# Autodesk Inventor assembly: Drive2
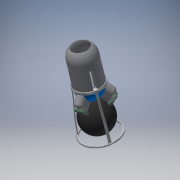
[picture p0: Inventor's stored thumbnail of the model, 180x180]
Saved by Autodesk Inventor 2019.1 (Build 231200000, 200)
## iProperties
Created: 2018-06-30
Part Number: Drive2
Material: Generisch
Document SubType Name: Assembly
Designer: JochenAlt
Author: JochenAlt
## Documents named in this file (10)
- D:\Projects\Ondine\CAD\Drive.iam
- D:\Projects\Ondine\CAD\Sphere.ipt
- D:\Projects\Ondine\CAD\DriveChain.iam
- D:\Projects\Ondine\CAD\Spindle\SpindleWithGear.ipt
- D:\Projects\Ondine\CAD\Spindle\Spindle.ipt
- D:\Projects\Ondine\CAD\Bearings\W 61700 X-2RS1.iam
- D:\Projects\Ondine\CAD\SpindleMotor.iam
- D:\Projects\Ondine\CAD\PCB\ControllerPCBHolder.ipt
- D:\Projects\Ondine\CAD\PCB\MotorController.ipt
- D:\Projects\Ondine\CAD\Form.iam
## Components (18 placed, 8 different names)
1. Sphere:1 — Passend:38, Passend:61, Passend:121, Passend:122
2. DriveChain:1 [sub-assembly] — Passend:61, Passend:95, Passend:103, Passend:104, Passend:105, Passend:110, Passend:115, Passend:121, Passend:122, Passend:127, Passend:130
3. DriveChain:2 [sub-assembly] — Passend:84, Passend:87, Passend:95, Passend:99, Passend:109, Passend:110, Passend:111, Passend:112, Passend:116
4. DriveChain:3 [sub-assembly] — Passend:89, Passend:93, Passend:103, Passend:104, Passend:111, Passend:113, Passend:128
5. Spindle:1 — Passend:66, Passend:72, Passend:77, Fluchtend:1
6. Spindle:2 — Passend:67, Passend:75, Passend:76, Passend:93
7. Spindle:3 — Passend:73, Passend:114, Passend:117, Passend:129
8. W 61700 X-2RS1:1 [sub-assembly] — Passend:66, Passend:112
9. W 61700 X-2RS1:2 [sub-assembly]
10. W 61700 X-2RS1:3 [sub-assembly] — Passend:67, Passend:113
11. W 61700 X-2RS1:4 [sub-assembly] — Passend:72, Passend:77, Passend:87, Passend:109
12. W 61700 X-2RS1:5 [sub-assembly] — Passend:75, Passend:76, Passend:89
13. W 61700 X-2RS1:6 [sub-assembly] — Passend:73, Passend:116, Passend:117
14. SpindleMotor:1 [sub-assembly] — Passend:84, Fluchtend:1
15. PCBHolder:1 — Passend:99, Passend:105, Passend:125, Passend:126, Passend:127, Passend:128
16. MotorController:1 — Passend:125, Passend:126
17. W 61700 X-2RS1:7 [sub-assembly] — Passend:114, Passend:115
18. Form:1 [sub-assembly] — Passend:129, Passend:130
## Relationships (36: Mate 35, Flush 1)
- Passend:38 [Mate]: Sphere:1
- Passend:61 [Mate] (89 mm): Sphere:1 ↔ DriveChain:1
- Passend:66 [Mate]: Spindle:1 ↔ W 61700 X-2RS1:1
- Passend:67 [Mate]: Spindle:2 ↔ W 61700 X-2RS1:3
- Passend:72 [Mate]: Spindle:1 ↔ W 61700 X-2RS1:4
- Passend:73 [Mate]: Spindle:3 ↔ W 61700 X-2RS1:6
- Passend:75 [Mate]: Spindle:2 ↔ W 61700 X-2RS1:5
- Passend:76 [Mate]: Spindle:2 ↔ W 61700 X-2RS1:5
- Passend:77 [Mate]: Spindle:1 ↔ W 61700 X-2RS1:4
- Passend:84 [Mate]: DriveChain:2 ↔ SpindleMotor:1
- Fluchtend:1 [Flush]: Spindle:1 ↔ SpindleMotor:1
- Passend:87 [Mate]: DriveChain:2 ↔ W 61700 X-2RS1:4
- Passend:89 [Mate]: DriveChain:3 ↔ W 61700 X-2RS1:5
- Passend:93 [Mate]: DriveChain:3 ↔ Spindle:2
- Passend:95 [Mate]: DriveChain:1 ↔ DriveChain:2
- Passend:99 [Mate]: DriveChain:2 ↔ PCBHolder:1
- Passend:103 [Mate]: DriveChain:1 ↔ DriveChain:3
- Passend:104 [Mate]: DriveChain:1 ↔ DriveChain:3
- Passend:105 [Mate]: DriveChain:1 ↔ PCBHolder:1
- Passend:109 [Mate]: DriveChain:2 ↔ W 61700 X-2RS1:4
- Passend:110 [Mate]: DriveChain:1 ↔ DriveChain:2
- Passend:111 [Mate]: DriveChain:2 ↔ DriveChain:3
- Passend:112 [Mate]: DriveChain:2 ↔ W 61700 X-2RS1:1
- Passend:113 [Mate]: DriveChain:3 ↔ W 61700 X-2RS1:3
- Passend:114 [Mate]: Spindle:3 ↔ W 61700 X-2RS1:7
- Passend:115 [Mate]: DriveChain:1 ↔ W 61700 X-2RS1:7
- Passend:116 [Mate]: DriveChain:2 ↔ W 61700 X-2RS1:6
- Passend:117 [Mate]: Spindle:3 ↔ W 61700 X-2RS1:6
- Passend:121 [Mate]: Sphere:1 ↔ DriveChain:1
- Passend:122 [Mate] (-302 mm): Sphere:1 ↔ DriveChain:1
- Passend:125 [Mate]: PCBHolder:1 ↔ MotorController:1
- Passend:126 [Mate]: PCBHolder:1 ↔ MotorController:1
- Passend:127 [Mate]: DriveChain:1 ↔ PCBHolder:1
- Passend:128 [Mate]: DriveChain:3 ↔ PCBHolder:1
- Passend:129 [Mate]: Spindle:3 ↔ Form:1
- Passend:130 [Mate]: DriveChain:1 ↔ Form:1
